# Autodesk Inventor assembly: Assembly2
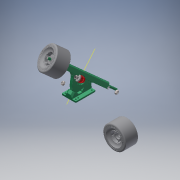
[picture p0: Inventor's stored thumbnail of the model, 180x180]
Saved by Autodesk Inventor 2018 (Build 220112000, 112)
## iProperties
Created: 2017-09-11
Part Number: Assembly2
Document SubType Name: Assembly
Designer: Rus
Author: Rus
## Documents named in this file (6)
- C:\Users\Rus\Documents\3D Models\Electric Longboard\Assembly2.iam
- C:\Users\Rus\Documents\3D Models\Electric Longboard\Trucks\50_CAL\50cal_truck.iam
- C:\Users\Rus\Documents\3D Models\Electric Longboard\Wheels\90mm_wheel_asm.iam
- C:\Users\Rus\Documents\3D Models\Electric Longboard\Trucks\50_CAL\608-bearing.ipt
- C:\Users\Rus\Documents\3D Models\Electric Longboard\Trucks\50_CAL\washer.ipt
- C:\Users\Rus\Documents\3D Models\Electric Longboard\Trucks\50_CAL\Axle-nut.ipt
## Components (8 placed, 5 different names)
1. 50cal_truck:1 [sub-assembly] — Insert:5
2. 90mm_wheel_asm:1 [sub-assembly] — Insert:1, Insert:2
3. 90mm_wheel_asm:2 [sub-assembly]
4. 608-bearing:1 — Insert:2, Insert:4
5. washer:1 — Insert:3
6. Axle-nut:1
7. 608-bearing:2 — Insert:1, Insert:3
8. washer:2 — Insert:4, Insert:5
## Relationships (5: Insert 5)
- Insert:1: 90mm_wheel_asm:1 ↔ 608-bearing:2
- Insert:2: 90mm_wheel_asm:1 ↔ 608-bearing:1
- Insert:3: washer:1 ↔ 608-bearing:2
- Insert:4: 608-bearing:1 ↔ washer:2
- Insert:5: 50cal_truck:1 ↔ washer:2
